# Autodesk Inventor assembly: Ball Bearing
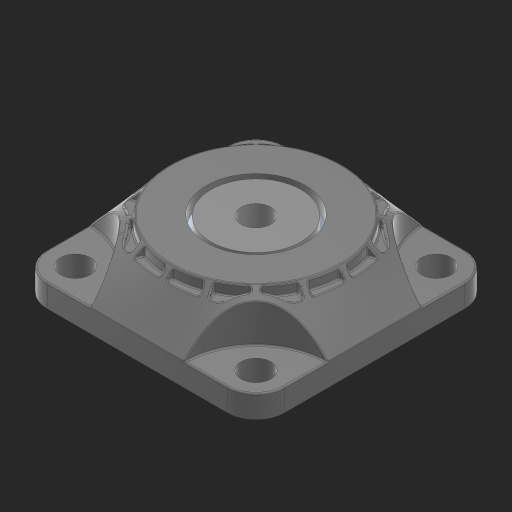
[picture p0: Inventor's stored thumbnail of the model, 512x512]
Saved by Autodesk Inventor 2023 (Build 270158000, 158)
## iProperties
Created: 2022-08-18
Part Number: Ball Bearing
Document SubType Name: Assembly
Designer: ylu12
Author: ylu12
## Documents named in this file (5)
- C:\Users\ylu12\Documents\GitHub\VEX-CAD-Inventor\Motion\Ball Bearing\Ball Bearing\Ball Bearing, Circle.iam
- C:\Users\ylu12\Documents\GitHub\VEX-CAD-Inventor\Motion\Ball Bearing\Reference Files\Ball Bearing Housing.ipt
- C:\Users\ylu12\Documents\GitHub\VEX-CAD-Inventor\Motion\Ball Bearing\Reference Files\Ball Bearing.ipt
- C:\Users\ylu12\Documents\GitHub\VEX-CAD-Inventor\Motion\Ball Bearing\Reference Files\Ball Bearing Circle Insert.ipt
- C:\Users\ylu12\Documents\GitHub\VEX-CAD-Inventor\Motion\Ball Bearing\Ball Bearing.iam
## Components (3 placed, 3 different names)
1. Ball Bearing Housing:1 — Mate:1, Mate:2
2. Ball Bearing:1 — Mate:1, Mate:2, Insert:1
3. Ball Bearing Circle Insert:1 — Insert:1
## Relationships (3: Mate 2, Insert 1)
- Mate:1: Ball Bearing Housing:1 ↔ Ball Bearing:1
- Mate:2: Ball Bearing Housing:1 ↔ Ball Bearing:1
- Insert:1: Ball Bearing:1 ↔ Ball Bearing Circle Insert:1
